# Autodesk Inventor assembly: AdeptOne
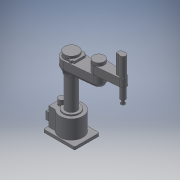
[picture p0: Inventor's stored thumbnail of the model, 180x180]
Saved by Autodesk Inventor 2016 (Build 200138000, 138)
## iProperties
Created: 2015-12-17
Part Number: AdeptOne
Document SubType Name: Assembly
Designer: ajshort
Author: ajshort
## Documents named in this file (5)
- C:\Users\ajshort\Documents\Inventor\AdeptOne\AdeptOne.iam
- C:\Users\ajshort\Documents\Inventor\AdeptOne\Base.ipt
- C:\Users\ajshort\Documents\Inventor\AdeptOne\1.ipt
- C:\Users\ajshort\Documents\Inventor\AdeptOne\2.ipt
- C:\Users\ajshort\Documents\Inventor\AdeptOne\4.ipt
## Components (4 placed, 4 different names)
1. Base:1 — Mate:1, Mate:2
2. 1:1 — Mate:1, Mate:2, Mate:3, Mate:4
3. 2:1 — Mate:3, Mate:4, Mate:5
4. 4:1 — Mate:5
## Relationships (5: Mate 5)
- Mate:1: Base:1 ↔ 1:1
- Mate:2: Base:1 ↔ 1:1
- Mate:3: 1:1 ↔ 2:1
- Mate:4: 1:1 ↔ 2:1
- Mate:5: 2:1 ↔ 4:1
